# Autodesk Inventor assembly: Assembly1
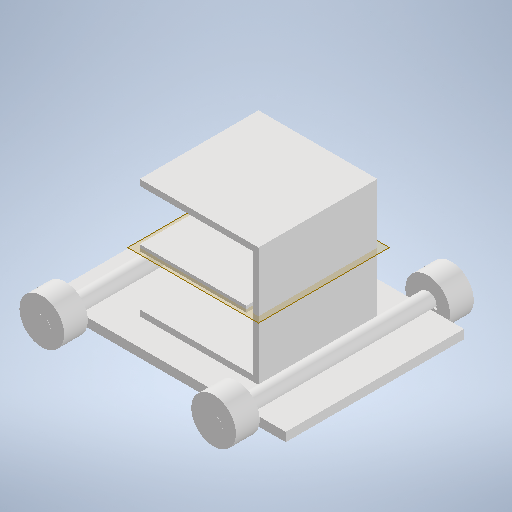
[picture p0: Inventor's stored thumbnail of the model, 512x512]
Saved by Autodesk Inventor 2025.3 (Build 293356030, 356C)
## iProperties
Created: 2026-06-23
Part Number: Assembly1
Document SubType Name: Assembly
Designer: user
Author: user
## Documents named in this file (5)
- C:\Docs\shcool\dojo\Flat\Assembly1.iam
- C:\Docs\shcool\dojo\Flat\Floor.ipt
- C:\Docs\shcool\dojo\Flat\Shaft.ipt
- C:\Docs\shcool\dojo\Flat\wheel.ipt
- C:\Docs\shcool\dojo\Flat\Holstrer.ipt
## Components (8 placed, 4 different names)
1. Floor:1 — Mate:2, Flush:1, Flush:2, Mate:3, Mate:4
2. Shaft:1 — Mate:2, Flush:1, Insert:2, Insert:4
3. Shaft:2 — Flush:2, Mate:3, Insert:1, Insert:3
4. wheel:1 — Insert:1
5. wheel:2 — Insert:2
6. wheel:3 — Insert:3
7. wheel:4 — Insert:4
8. Holstrer:1 — Mate:4
## Relationships (9: Insert 4, Mate 3, Flush 2)
- Mate:2: Floor:1 ↔ Shaft:1
- Flush:1 (50 mm): Floor:1 ↔ Shaft:1
- Flush:2 (-50 mm): Floor:1 ↔ Shaft:2
- Mate:3: Floor:1 ↔ Shaft:2
- Insert:1: Shaft:2 ↔ wheel:1
- Insert:2: Shaft:1 ↔ wheel:2
- Insert:3: Shaft:2 ↔ wheel:3
- Insert:4: Shaft:1 ↔ wheel:4
- Mate:4: Floor:1 ↔ Holstrer:1
